# Autodesk Inventor assembly: 555_GearBox
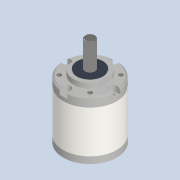
[picture p0: Inventor's stored thumbnail of the model, 180x180]
Saved by Autodesk Inventor 2021 (Build 250183000, 183)
## iProperties
Created: 2021-08-07
Part Number: 555_GearBox
Document SubType Name: Assembly
Designer: Hagihara Yuya
Mass: 149 g
Surface Area: 132.165 cm^2
Volume: 20.226 cm^3
Author: Hagihara Yuya
## Documents named in this file (6)
- C:\Users\Hagihara Yuya\Documents\GrabCAD\NHK2021\BasicParts\よく使う部品（萩原）\Motor\555\555_GearBox.iam
- C:\Users\Hagihara Yuya\Documents\GrabCAD\NHK2021\BasicParts\よく使う部品（萩原）\Motor\555\555_GearBox_Flange.ipt
- C:\Users\Hagihara Yuya\Documents\GrabCAD\NHK2021\BasicParts\よく使う部品（萩原）\Motor\555\555_GearBox_Body.ipt
- C:\Users\Hagihara Yuya\Documents\GrabCAD\NHK2021\BasicParts\よく使う部品（萩原）\Motor\555\555_GearBox_FrontCover.ipt
- C:\Users\Hagihara Yuya\Documents\GrabCAD\NHK2021\BasicParts\よく使う部品（萩原）\Motor\555\555_GearBox_FrontCircle.ipt
- C:\Users\Hagihara Yuya\Documents\GrabCAD\NHK2021\BasicParts\よく使う部品（萩原）\Motor\555\555_GearBox_Shaft.ipt
## Components (5 placed, 5 different names)
1. 555_GearBox_Flange:1 — リジッド:1
2. 555_GearBox_Body:1 — リジッド:1, 回転:1, フラッシュ:1
3. 555_GearBox_FrontCover:1 — 回転:1, フラッシュ:1, 回転:2, 回転:3
4. 555_GearBox_FrontCircle:1 — 回転:2
5. 555_GearBox_Shaft:1 — 回転:3
## Relationships (5: RevoluteJoint 3, WeldJoint 1, Flush 1)
- リジッド:1 [WeldJoint]: 555_GearBox_Flange:1 ↔ 555_GearBox_Body:1
- 回転:1 [RevoluteJoint]: 555_GearBox_Body:1 ↔ 555_GearBox_FrontCover:1
- フラッシュ:1 [Flush]: 555_GearBox_Body:1 ↔ 555_GearBox_FrontCover:1
- 回転:2 [RevoluteJoint]: 555_GearBox_FrontCover:1 ↔ 555_GearBox_FrontCircle:1
- 回転:3 [RevoluteJoint]: 555_GearBox_FrontCover:1 ↔ 555_GearBox_Shaft:1
